# Autodesk Inventor assembly: New Back Board Assembly
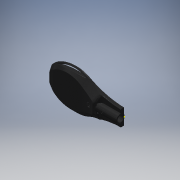
[picture p0: Inventor's stored thumbnail of the model, 180x180]
Saved by Autodesk Inventor 2018 (Build 220112000, 112)
## iProperties
Created: 2018-04-07
Part Number: New Back Board Assembly
Document SubType Name: Assembly
Designer: Cole
Author: Cole
## Documents named in this file (3)
- P:\IED\SchoolCAD\ReverseEngineering\New Back Board Assembly.iam
- P:\IED\SchoolCAD\ReverseEngineering\Back Board Cover.ipt
- P:\IED\SchoolCAD\ReverseEngineering\New Back Board.ipt
## Components (2 placed, 2 different names)
1. Back Board Cover:1 — Mate:1, Mate:2, Mate:3
2. New Back Board:1 — Mate:1, Mate:2, Mate:3
## Relationships (3: Mate 3)
- Mate:1: Back Board Cover:1 ↔ New Back Board:1
- Mate:2: Back Board Cover:1 ↔ New Back Board:1
- Mate:3: Back Board Cover:1 ↔ New Back Board:1
